# Autodesk Inventor assembly: SimulationWheelAssembly
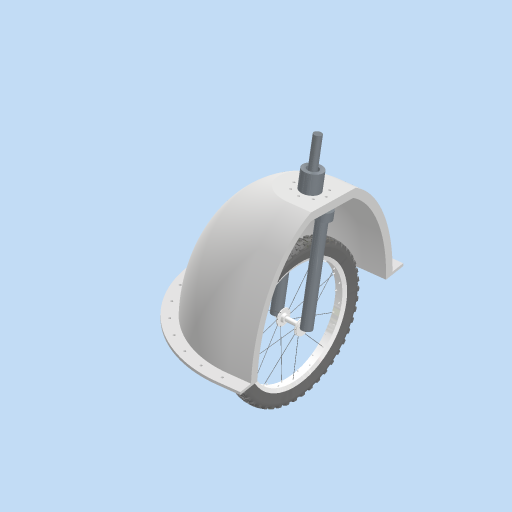
[picture p0: Inventor's stored thumbnail of the model, 512x512]
Saved by Autodesk Inventor 2023 (Build 270158000, 158)
## iProperties
Created: 2026-03-22
Part Number: SimulationWheelAssembly
Document SubType Name: Assembly
Designer: Nathann
Author: Nathann
## Documents named in this file (4)
- C:\Users\Nathann\ClawdDrive\Objet3D\neodrive\neodrive-cad-ergonomic-v1\SimulationWheelAssembly.iam
- C:\Users\Nathann\ClawdDrive\Objet3D\neodrive\neodrive-cad-ergonomic-v1\eggshellCorePrintedLeft.ipt
- C:\Users\Nathann\ClawdDrive\Objet3D\neodrive\neodrive-cad-ergonomic-v1\neodrive-cad-ergonomic-v1-AssemblyWheelAndFork005.ipt
- C:\Users\Nathann\ClawdDrive\Objet3D\neodrive\neodrive-cad-ergonomic-v1\neodrive-cad-ergonomic-v1-AssemblyForkHardpoint001.ipt
## Components (3 placed, 3 different names)
1. eggshellCorePrintedLeft:1
2. neodrive-cad-ergonomic-v1-AssemblyWheelAndFork005:1
3. neodrive-cad-ergonomic-v1-AssemblyForkHardpoint001:1
## Relationships (2: Insert 2)
- [Insert]: eggshellCorePrintedLeft:1 ↔ neodrive-cad-ergonomic-v1-AssemblyForkHardpoint001:1
- [Insert]: neodrive-cad-ergonomic-v1-AssemblyWheelAndFork005:1 ↔ neodrive-cad-ergonomic-v1-AssemblyForkHardpoint001:1
